# Autodesk Inventor assembly: UpperArmLeft
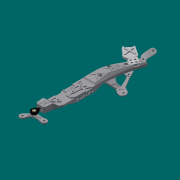
[picture p0: Inventor's stored thumbnail of the model, 180x180]
Saved by Autodesk Inventor 2015 SP1 (Build 190203100, 203)
## iProperties
Created: 2016-10-01
Part Number: UpperArmLeft
Document SubType Name: Assembly
Designer: Val
Author: Val
## Documents named in this file (7)
- C:\Users\Val\Desktop\ExoGit\elysium-max-exoskeleton\src\Assemblies\UpperArmLeft.iam
- C:\Users\Val\Desktop\ExoGit\elysium-max-exoskeleton\src\UpperArmLeft.ipt
- C:\Users\Val\Desktop\ExoGit\elysium-max-exoskeleton\src\UpperArmShoulderLeft.ipt
- C:\Users\Val\Desktop\ExoGit\elysium-max-exoskeleton\src\UpperArmTricepLeft.ipt
- C:\Users\Val\Desktop\ExoGit\elysium-max-exoskeleton\src\External\Bearing.iam
- C:\Users\Val\Desktop\ExoGit\elysium-max-exoskeleton\src\UpperArmConnectorLeft.ipt
- C:\Users\Val\Desktop\ExoGit\elysium-max-exoskeleton\src\ElbowSubConnectorLeft.ipt
## Components (6 placed, 6 different names)
1. UpperArmLeft:1 — Mate:1, Mate:2, Mate:3, Mate:4, Mate:5, Mate:6, Mate:7, Flush:1, Angle:1, Mate:8, Mate:9, Flush:2
2. UpperArmShoulderLeft:1 — Mate:1, Mate:2, Mate:3
3. UpperArmTricepLeft:1 — Mate:4, Mate:5, Mate:6
4. Bearing:1 [sub-assembly] — Mate:7, Flush:1, Angle:1, Mate:8, Mate:10, Mate:11
5. UpperArmTwistConnectorLeft:1 — Mate:9, Flush:2
6. ElbowSubConnectorLeft:1 — Mate:10, Mate:11
## Relationships (14: Mate 11, Flush 2, Angle 1)
- Mate:1: UpperArmLeft:1 ↔ UpperArmShoulderLeft:1
- Mate:2: UpperArmLeft:1 ↔ UpperArmShoulderLeft:1
- Mate:3: UpperArmLeft:1 ↔ UpperArmShoulderLeft:1
- Mate:4: UpperArmLeft:1 ↔ UpperArmTricepLeft:1
- Mate:5: UpperArmLeft:1 ↔ UpperArmTricepLeft:1
- Mate:6: UpperArmLeft:1 ↔ UpperArmTricepLeft:1
- Mate:7: UpperArmLeft:1 ↔ Bearing:1
- Flush:1 (-15 mm): UpperArmLeft:1 ↔ Bearing:1
- Angle:1 (0 deg): UpperArmLeft:1 ↔ Bearing:1
- Mate:8 (-15 mm): UpperArmLeft:1 ↔ Bearing:1
- Mate:9: UpperArmLeft:1 ↔ UpperArmTwistConnectorLeft:1
- Flush:2: UpperArmLeft:1 ↔ UpperArmTwistConnectorLeft:1
- Mate:10: Bearing:1 ↔ ElbowSubConnectorLeft:1
- Mate:11: Bearing:1 ↔ ElbowSubConnectorLeft:1
